# Autodesk Inventor assembly: Assembly1
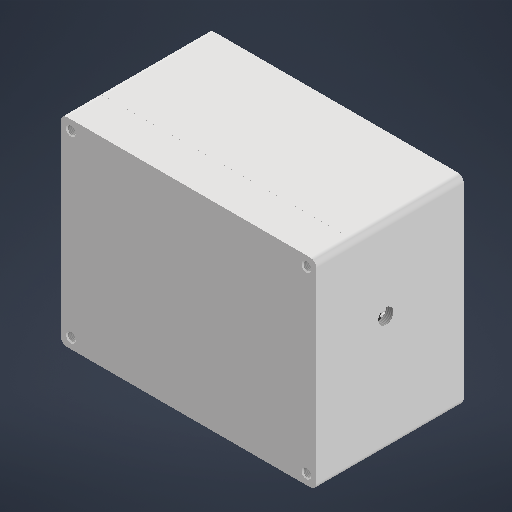
[picture p0: Inventor's stored thumbnail of the model, 512x512]
Saved by Autodesk Inventor 2027.1 (Build 311270010, 270A)
## iProperties
Created: 2026-09-14
Part Number: Assembly1
Document SubType Name: Assembly
Designer: LENOVO
Author: LENOVO
## Documents named in this file (7)
- C:\Users\LENOVO\OneDrive\Documents\PROJECK RISET\BOX_PANEL\Assembly1.iam
- C:\Users\LENOVO\Downloads\ESP32-DevkitC32U\ESP32-DevkitC32U.ipt
- C:\Users\LENOVO\Downloads\HI-LINK HLK-PM01 3W 5VDC v1\HI-LINK HLK-PM01 3W 5VDC v1.ipt
- C:\Users\LENOVO\OneDrive\Documents\TTL_TO_RS485.ipt
- C:\Users\LENOVO\OneDrive\Documents\dudukan_hi-link.ipt
- C:\Users\LENOVO\OneDrive\Documents\BOX_PANEL.ipt
- C:\Users\LENOVO\OneDrive\Documents\TUTUP_BOX1.ipt
## Components (6 placed, 6 different names)
1. ESP32-DevkitC32U:1
2. HI-LINK HLK-PM01 3W 5VDC v1:2 — Flush:1
3. TTL_TO_RS485:1
4. dudukan_hi-link:1 — Flush:1
5. BOX_PANEL:1 — Flush:2, Flush:3
6. TUTUP_BOX1:1 — Flush:2, Flush:3
## Relationships (3: Flush 3)
- Flush:1: HI-LINK HLK-PM01 3W 5VDC v1:2 ↔ dudukan_hi-link:1
- Flush:2: BOX_PANEL:1 ↔ TUTUP_BOX1:1
- Flush:3: BOX_PANEL:1 ↔ TUTUP_BOX1:1
